# Autodesk Inventor assembly: diy-rail-370-assembly
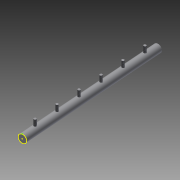
[picture p0: Inventor's stored thumbnail of the model, 180x180]
Saved by Autodesk Inventor 2014 (Build 180170000, 170)
## iProperties
Created: 2014-08-19
Part Number: diy-rail-370-assembly
Document SubType Name: Assembly
Designer: Matthew
Author: Matthew
## Documents named in this file (3)
- C:\Users\Matthew\Documents\GitHub\CNC Mill\diy-rail-370\diy-rail-370-assembly.iam
- C:\Users\Matthew\Documents\GitHub\CNC Mill\diy-rail_370mm.ipt
- C:\Users\Matthew\Documents\GitHub\CNC Mill\diy-rail-370\4-20_screw.ipt
## Components (7 placed, 2 different names)
1. diy-rail_370mm:1 — Insert:1, Insert:2, Insert:3, Insert:4, Insert:5, Insert:6
2. 4-20_screw:1 — Insert:2
3. 4-20_screw:2 — Insert:6
4. 4-20_screw:3 — Insert:3
5. 4-20_screw:4 — Insert:4
6. 4-20_screw:5 — Insert:5
7. 4-20_screw:6 — Insert:1
## Relationships (6: Insert 6)
- Insert:1: diy-rail_370mm:1 ↔ 4-20_screw:6
- Insert:2: diy-rail_370mm:1 ↔ 4-20_screw:1
- Insert:3: diy-rail_370mm:1 ↔ 4-20_screw:3
- Insert:4: diy-rail_370mm:1 ↔ 4-20_screw:4
- Insert:5: diy-rail_370mm:1 ↔ 4-20_screw:5
- Insert:6: diy-rail_370mm:1 ↔ 4-20_screw:2
